# Autodesk Inventor assembly: ASY SLM 1210 MAIN FRAME
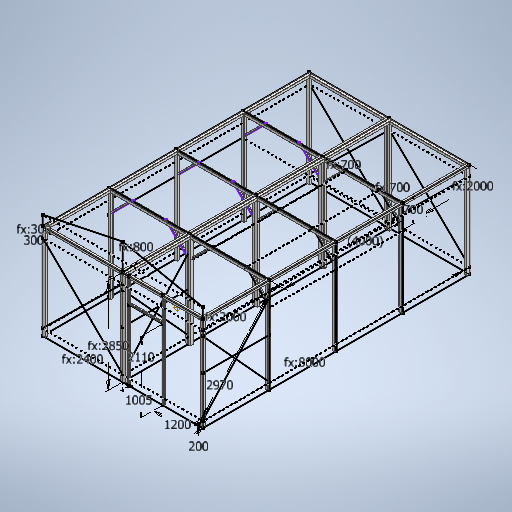
[picture p0: Inventor's stored thumbnail of the model, 512x512]
Saved by Autodesk Inventor 2025.4 (Build 294407000, 407)
## iProperties
_SolveAssemblyDoc: Frame Generator Solve Assembly
_Version: 25.0.0
Created: 2026-01-26
Part Number: ASY SLM 1210 MAIN FRAME
Document SubType Name: Assembly
Designer: admin
Author: admin
## Documents named in this file (3)
- C:\Users\admin\Documents\Inventor\SLM-Salemal\ASY SLM 1210 MAIN FRAME.iam
- C:\Users\admin\Documents\Inventor\SLM-Salemal\PNS-1100 FRAME OLD sketch.ipt
- C:\Users\admin\Documents\Inventor\SLM-Salemal\ASY SLM 1210 MAIN FRAME\Frame\Frame 1769424024765.iam
## Components (2 placed, 2 different names)
1. PNS-1121 FRAME OLD sketch:1 — Flush:1, Mate:1, Flush:2
2. Frame 1769424024765:1 [sub-assembly]
## Relationships (3: Flush 2, Mate 1)
- Flush:1: PNS-1121 FRAME OLD sketch:1
- Mate:1: PNS-1121 FRAME OLD sketch:1
- Flush:2: PNS-1121 FRAME OLD sketch:1
